# Autodesk Inventor assembly: holder_with_battery
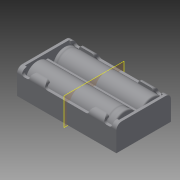
[picture p0: Inventor's stored thumbnail of the model, 180x180]
Saved by Autodesk Inventor 2014 (Build 180170000, 170)
## iProperties
Created: 2013-06-25
Part Number: holder_with_battery
Document SubType Name: Assembly
Designer: Felix
Author: Felix
## Documents named in this file (3)
- C:\Users\Felix\Desktop\Beep\Hardware\3D-CAD\battery_holder\holder_with_batteries_18650.iam
- C:\Users\Felix\Desktop\Beep\Hardware\3D-CAD\battery_holder\battery_18650.ipt
- C:\Users\Felix\Desktop\Beep\Hardware\3D-CAD\battery_holder\holder_18650.ipt
## Components (3 placed, 2 different names)
1. battery_18650:1 — Passend:1
2. battery_18650:2 — Passend:2
3. holder_18650:1 — Passend:1, Passend:2
## Relationships (2: Mate 2)
- Passend:1 [Mate]: battery_18650:1 ↔ holder_18650:1
- Passend:2 [Mate]: battery_18650:2 ↔ holder_18650:1
